# Autodesk Inventor assembly: Cahyo
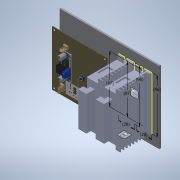
[picture p0: Inventor's stored thumbnail of the model, 180x180]
Saved by Autodesk Inventor 2020 (Build 240168000, 168)
## iProperties
Created: 2021-04-23
Part Number: Cahyo
Document SubType Name: Assembly
Designer: Administrator
Title: Cahyo v18
Author: Administrator
## Documents named in this file (4)
- E:\Github\Nawaytes\TM-alat uji tekan\ECAD\render\Cahyo v18\Cahyo.iam
- E:\Github\Nawaytes\TM-alat uji tekan\ECAD\render\Cahyo v18\PCB Component.iam
- E:\Github\Nawaytes\TM-alat uji tekan\MCAD\Akrilik.ipt
- E:\junk\tb-6600-driver-1.snapshot.1\driver tb6600.ipt
## Components (4 placed, 3 different names)
1. PCB Component:1 [sub-assembly]
2. Akrilik:1 — Mate:1, Mate:2
3. driver tb6600:3 — Mate:1, Flush:1
4. driver tb6600:4 — Mate:2, Flush:1
## Relationships (3: Mate 2, Flush 1)
- Mate:1: Akrilik:1 ↔ driver tb6600:3
- Mate:2: Akrilik:1 ↔ driver tb6600:4
- Flush:1: driver tb6600:3 ↔ driver tb6600:4
